# Autodesk Inventor assembly: Mold Design33
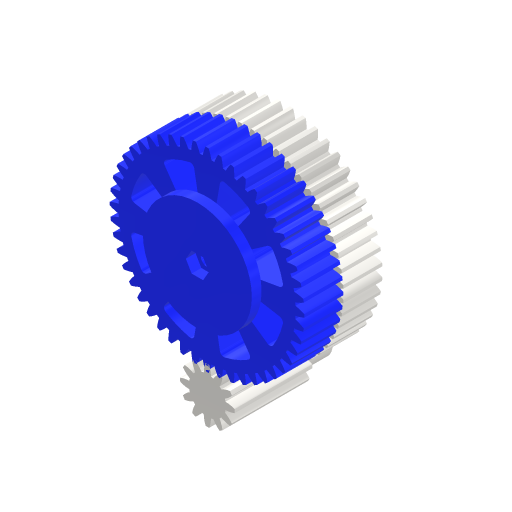
[picture p0: Inventor's stored thumbnail of the model, 512x512]
Saved by Autodesk Inventor 2024 (Build 280153000, 153)
## iProperties
Created: 2023-07-11
Part Number: Mold Design33
Document SubType Name: Assembly
Designer: ferna
Author: ferna
## Documents named in this file (3)
- C:\Users\ferna\OneDrive - Universidad Católica de Chile\Bocas\RobotFlautista\Mold Design1\Mold Design33.iam
- C:\Users\ferna\OneDrive - Universidad Católica de Chile\Bocas\RobotFlautista\Mold Design1\Mold Design33\Design Accelerator\Spur Gears1.iam
- C:\Users\ferna\Documents\Modelos3D\tapaComandante3.ipt
## Components (2 placed, 2 different names)
1. Spur Gears:1 [sub-assembly] — Mate:1
2. tapaComandante3:1 — Mate:1
## Relationships (1: Mate 1)
- Mate:1: Spur Gears:1 ↔ tapaComandante3:1
